# Autodesk Inventor assembly: juki-head-assembly
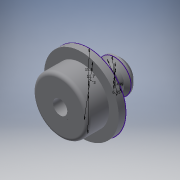
[picture p0: Inventor's stored thumbnail of the model, 180x180]
Saved by Autodesk Inventor 2017 (Build 210142000, 142)
## iProperties
Created: 2026-03-25
Part Number: juki-head-assembly
Document SubType Name: Assembly
Designer: a
Author: a
## Documents named in this file (3)
- C:\Users\a\Documents\the-claw-pnp\juki-head-assembly.iam
- C:\Users\a\Documents\the-claw-pnp\juki-mount.ipt
- C:\Users\a\Documents\the-claw-pnp\juki-nozzle-base.ipt
## Components (2 placed, 2 different names)
1. juki-mount:1 — Mate:1, Mate:2
2. juki-nozzle-base:1 — Mate:1, Mate:2
## Relationships (2: Mate 2)
- Mate:1: juki-mount:1 ↔ juki-nozzle-base:1
- Mate:2: juki-mount:1 ↔ juki-nozzle-base:1
